# Autodesk Inventor assembly: Intake
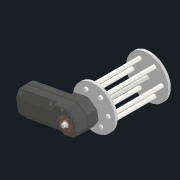
[picture p0: Inventor's stored thumbnail of the model, 180x180]
Saved by Autodesk Inventor 2022 (Build 260153000, 153)
## iProperties
Created: 2021-12-07
Part Number: Intake
Document SubType Name: Assembly
Designer: divid
Author: divid
## Documents named in this file (5)
- C:\Users\divid\Documents\GitHub\ComputerAidedDesign\2021-22\FTC\#13822 Robovikes\Intake\Intake.iam
- C:\Users\divid\Documents\GitHub\ComputerAidedDesign\2021-22\FTC\#13822 Robovikes\Intake\Input _Ring.ipt
- C:\Users\divid\Documents\GitHub\ComputerAidedDesign\2021-22\FTC\#13822 Robovikes\Intake\5mm x 90mm Hex Shaft - 4 Pack.ipt
- C:\Users\divid\Documents\GitHub\ComputerAidedDesign\2021-22\FTC\#13822 Robovikes\Intake\5mm x 135mm Hex Shaft - 4 Pack.ipt
- C:\Users\divid\Documents\GitHub\ComputerAidedDesign\2021-22\FTC\#13822 Robovikes\Intake\Core Hex Motor.ipt
## Components (10 placed, 4 different names)
1. Input _Ring:1 — Flush:1, Flush:2, Mate:1, Mate:2, Mate:3, Mate:5, Mate:6, Mate:7, Mate:8, Mate:9, Mate:10
2. Input _Ring:2 — Flush:1, Flush:2, Mate:4
3. 5mm x 90mm Hex Shaft - 4 Pack:1 — Mate:1, Mate:2
4. 5mm x 90mm Hex Shaft - 4 Pack:2 — Mate:3, Mate:4
5. 5mm x 90mm Hex Shaft - 4 Pack:3 — Mate:5, Mate:6
6. 5mm x 90mm Hex Shaft - 4 Pack:4 — Mate:7, Mate:8
7. 5mm x 90mm Hex Shaft - 4 Pack:5
8. 5mm x 90mm Hex Shaft - 4 Pack:6
9. 5mm x 135mm Hex Shaft - 4 Pack:1 — Mate:9, Mate:10, Mate:11, Mate:12
10. Core Hex Motor:1 — Mate:11, Mate:12
## Relationships (14: Mate 12, Flush 2)
- Flush:1: Input _Ring:1 ↔ Input _Ring:2
- Flush:2: Input _Ring:1 ↔ Input _Ring:2
- Mate:1: Input _Ring:1 ↔ 5mm x 90mm Hex Shaft - 4 Pack:1
- Mate:2: Input _Ring:1 ↔ 5mm x 90mm Hex Shaft - 4 Pack:1
- Mate:3: Input _Ring:1 ↔ 5mm x 90mm Hex Shaft - 4 Pack:2
- Mate:4: Input _Ring:2 ↔ 5mm x 90mm Hex Shaft - 4 Pack:2
- Mate:5: Input _Ring:1 ↔ 5mm x 90mm Hex Shaft - 4 Pack:3
- Mate:6: Input _Ring:1 ↔ 5mm x 90mm Hex Shaft - 4 Pack:3
- Mate:7: Input _Ring:1 ↔ 5mm x 90mm Hex Shaft - 4 Pack:4
- Mate:8: Input _Ring:1 ↔ 5mm x 90mm Hex Shaft - 4 Pack:4
- Mate:9: Input _Ring:1 ↔ 5mm x 135mm Hex Shaft - 4 Pack:1
- Mate:10: Input _Ring:1 ↔ 5mm x 135mm Hex Shaft - 4 Pack:1
- Mate:11: 5mm x 135mm Hex Shaft - 4 Pack:1 ↔ Core Hex Motor:1
- Mate:12: 5mm x 135mm Hex Shaft - 4 Pack:1 ↔ Core Hex Motor:1
